# Autodesk Inventor assembly: Assembly7
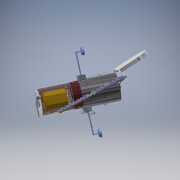
[picture p0: Inventor's stored thumbnail of the model, 180x180]
Saved by Autodesk Inventor 2018 (Build 220112000, 112)
## iProperties
Created: 2021-03-18
Part Number: Assembly7
Document SubType Name: Assembly
Designer: dell
Author: dell
## Documents named in this file (8)
- D:\Autodesk\Projects\C-C\a1\ES101 GROUP-13 PROJECT\FINAL MODEL\Hubble Space Telescope.iam
- D:\Autodesk\Projects\C-C\a1\ES101 GROUP-13 PROJECT\INDIVIDUAL WORK\Kush\Resolved parts\Assembly_panel.iam
- D:\Autodesk\Projects\C-C\a1\ES101 GROUP-13 PROJECT\FINAL MODEL\Resolved files\Assembly6.iam
- D:\Autodesk\Projects\C-C\a1\ES101 GROUP-13 PROJECT\INDIVIDUAL WORK\Kush\Aparture_door.ipt
- D:\Autodesk\Projects\C-C\a1\ES101 GROUP-13 PROJECT\INDIVIDUAL WORK\Nitesh\SupportingRod.ipt
- D:\Autodesk\Projects\C-C\a1\ES101 GROUP-13 PROJECT\INDIVIDUAL WORK\Nitin\PrimaryMirror.iam
- D:\Autodesk\Projects\C-C\a1\ES101 GROUP-13 PROJECT\INDIVIDUAL WORK\Dishant\LGA.ipt
- D:\Autodesk\Projects\C-C\a1\ES101 GROUP-13 PROJECT\INDIVIDUAL WORK\Dishant\Resolved files\Derived HGA.ipt
## Components (13 placed, 7 different names)
1. Aparture_door:1 — Mate:1, Mate:2
2. Assembly6:1 [sub-assembly] — Mate:1, Mate:2, Mate:9, Mate:14, Mate:15, Mate:16, Mate:17, Flush:1, Flush:2, Mate:19, Mate:20, Mate:21, Mate:22, Mate:23, Mate:24, Mate:25, Mate:26, Mate:27, Mate:28, Mate:29, Mate:30
3. Assembly_panel:2 [sub-assembly] — Mate:4, Mate:6
4. SupportingRod:1 — Mate:4, Mate:5, Mate:6, Mate:7, Mate:8
5. SupportingRod:2 — Mate:5, Mate:7, Mate:8, Mate:9, Mate:16
6. Assembly_panel:3 [sub-assembly] — Mate:10, Mate:13
7. SupportingRod:3 — Mate:11, Mate:12, Mate:14, Mate:15
8. SupportingRod:4 — Mate:10, Mate:11, Mate:12, Mate:13
9. PrimaryMirror:1 [sub-assembly] — Mate:17, Mate:18
10. LGA:3 — Mate:19, Mate:20, Mate:23
11. LGA:4 — Mate:21, Mate:22, Mate:24
12. Derived HGA:1 — Mate:25, Mate:26, Mate:27
13. Derived HGA:2 — Mate:28, Mate:29, Mate:30
## Relationships (31: Mate 29, Flush 2)
- Mate:1: Aparture_door:1 ↔ Assembly6:1
- Mate:2: Aparture_door:1 ↔ Assembly6:1
- Mate:4: Assembly_panel:2 ↔ SupportingRod:1
- Mate:5: SupportingRod:1 ↔ SupportingRod:2
- Mate:6: Assembly_panel:2 ↔ SupportingRod:1
- Mate:7: SupportingRod:1 ↔ SupportingRod:2
- Mate:8: SupportingRod:1 ↔ SupportingRod:2
- Mate:9: Assembly6:1 ↔ SupportingRod:2
- Mate:10: Assembly_panel:3 ↔ SupportingRod:4
- Mate:11: SupportingRod:3 ↔ SupportingRod:4
- Mate:12: SupportingRod:3 ↔ SupportingRod:4
- Mate:13: Assembly_panel:3 ↔ SupportingRod:4
- Mate:14: Assembly6:1 ↔ SupportingRod:3
- Mate:15 (88 mm): Assembly6:1 ↔ SupportingRod:3
- Mate:16 (88 mm): Assembly6:1 ↔ SupportingRod:2
- Mate:17: Assembly6:1 ↔ PrimaryMirror:1
- Flush:1 (2 mm): Assembly6:1
- Mate:18: PrimaryMirror:1
- Flush:2: Assembly6:1
- Mate:19: Assembly6:1 ↔ LGA:3
- Mate:20 (145 mm): Assembly6:1 ↔ LGA:3
- Mate:21 (145 mm): Assembly6:1 ↔ LGA:4
- Mate:22: Assembly6:1 ↔ LGA:4
- Mate:23 (120 mm): Assembly6:1 ↔ LGA:3
- Mate:24 (120 mm): Assembly6:1 ↔ LGA:4
- Mate:25: Assembly6:1 ↔ Derived HGA:1
- Mate:26 (35 mm): Assembly6:1 ↔ Derived HGA:1
- Mate:27 (28 mm): Assembly6:1 ↔ Derived HGA:1
- Mate:28: Assembly6:1 ↔ Derived HGA:2
- Mate:29 (35 mm): Assembly6:1 ↔ Derived HGA:2
- Mate:30 (22 mm): Assembly6:1 ↔ Derived HGA:2
